# Autodesk Inventor assembly: 組合檔
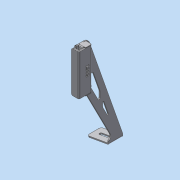
[picture p0: Inventor's stored thumbnail of the model, 180x180]
Saved by Autodesk Inventor 2020 (Build 240168000, 168)
## iProperties
Created: 2015-11-28
Part Number: 組合檔
Document SubType Name: Assembly
Designer: 設計製圖
Author: 設計製圖
## Documents named in this file (13)
- D:\資料庫\設計-3D產品\【May club 】\得利卡-車頂燈架\模型、圖面\車頂燈架-組合 - 複製.iam
- D:\資料庫\設計-3D產品\【May club 】\得利卡-車頂燈架\模型、圖面\吊架-長(R).ipt
- D:\資料庫\設計-3D產品\【May club 】\得利卡-車頂燈架\模型、圖面\概-膠條.ipt
- D:\資料庫\設計-3D產品\【May club 】\得利卡-車頂燈架\模型、圖面\概-泡棉墊(1).ipt
- D:\資料庫\設計-3D產品\【May club 】\得利卡-車頂燈架\模型、圖面\概-泡棉墊(3).ipt
- D:\資料庫\設計-3D產品\【 鐵蹄 】\------鐵蹄工廠素材------ -\拉帽-M8.ipt
- D:\資料庫\設計-3D產品\【May club 】\得利卡-車頂燈架\模型、圖面\焊接組件-1.ipt
- D:\資料庫\設計-3D產品\【May club 】\得利卡-車頂燈架\模型、圖面\焊接組件-3.ipt
- D:\資料庫\設計-3D產品\【May club 】\得利卡-車頂燈架\模型、圖面\概-泡棉墊(2).ipt
- D:\資料庫\設計-3D產品\【May club 】\得利卡-車頂燈架\模型、圖面\焊接組件-2.ipt
- D:\資料庫\設計-3D產品\材料庫\【螺絲】\止付螺絲\止付螺絲-M8-20.ipt
- D:\資料庫\設計-3D產品\【May club 】\得利卡-車頂燈架\模型、圖面\車身圖.ipt
- D:\資料庫\設計-3D產品\【May club 】\得利卡-車頂燈架\模型、圖面\吊架組件-ㄇ槽.ipt
## Components (14 placed, 12 different names)
1. 車身圖:1 — 貼合:33
2. 吊架組件-ㄇ槽:1 — 貼合:6, 齊平:2, 齊平:3, 貼合:8, 齊平:4, 貼合:17, 貼合:18, 貼合:24, 貼合:35, 貼合:36, 貼合:37, 貼合:38
3. 吊架-長(R):1 — 貼合:3, 貼合:4, 齊平:1, 貼合:18, 貼合:23, 貼合:25, 貼合:26, 貼合:28, 齊平:9, 齊平:10, 貼合:33
4. 焊接組件-1:1 — 貼合:29, 貼合:30, 齊平:11
5. 焊接組件-3:1 — 貼合:23, 貼合:24, 貼合:25, 貼合:26, 貼合:27, 齊平:7, 齊平:8
6. 焊接組件-2:1 — 貼合:28, 齊平:9, 齊平:10, 貼合:29, 貼合:30, 齊平:11
7. 拉帽-M8:1 — 齊平:6, 貼合:15, 貼合:17, 貼合:31, 貼合:35, 貼合:37
8. 拉帽-M8:2 — 齊平:6, 貼合:15, 貼合:32, 貼合:36, 貼合:38
9. 概-泡棉墊(2):1 — 貼合:27, 齊平:7, 齊平:8
10. 概-膠條:1 — 貼合:3, 貼合:4, 齊平:1
11. 概-泡棉墊(1):1 — 貼合:6, 齊平:2, 齊平:3, 貼合:9
12. 概-泡棉墊(3):1 — 貼合:8, 貼合:9, 齊平:4
13. 止付螺絲-M8-20:1 — 齊平:12, 貼合:31
14. 止付螺絲-M8-20:2 — 齊平:12, 貼合:32
## Relationships (34: Mate 23, Flush 11)
- 貼合:3 [Mate]: 吊架-長(R):1 ↔ 概-膠條:1
- 貼合:4 [Mate]: 吊架-長(R):1 ↔ 概-膠條:1
- 齊平:1 [Flush]: 吊架-長(R):1 ↔ 概-膠條:1
- 貼合:6 [Mate]: 吊架組件-ㄇ槽:1 ↔ 概-泡棉墊(1):1
- 齊平:2 [Flush]: 吊架組件-ㄇ槽:1 ↔ 概-泡棉墊(1):1
- 齊平:3 [Flush]: 吊架組件-ㄇ槽:1 ↔ 概-泡棉墊(1):1
- 貼合:8 [Mate]: 吊架組件-ㄇ槽:1 ↔ 概-泡棉墊(3):1
- 貼合:9 [Mate]: 概-泡棉墊(1):1 ↔ 概-泡棉墊(3):1
- 齊平:4 [Flush]: 吊架組件-ㄇ槽:1 ↔ 概-泡棉墊(3):1
- 齊平:6 [Flush]: 拉帽-M8:1 ↔ 拉帽-M8:2
- 貼合:15 [Mate]: 拉帽-M8:1 ↔ 拉帽-M8:2
- 貼合:17 [Mate]: 吊架組件-ㄇ槽:1 ↔ 拉帽-M8:1
- 貼合:18 [Mate]: 吊架組件-ㄇ槽:1 ↔ 吊架-長(R):1
- 貼合:23 [Mate]: 吊架-長(R):1 ↔ 焊接組件-3:1
- 貼合:24 [Mate]: 吊架組件-ㄇ槽:1 ↔ 焊接組件-3:1
- 貼合:25 [Mate]: 吊架-長(R):1 ↔ 焊接組件-3:1
- 貼合:26 [Mate]: 吊架-長(R):1 ↔ 焊接組件-3:1
- 貼合:27 [Mate]: 焊接組件-3:1 ↔ 概-泡棉墊(2):1
- 齊平:7 [Flush]: 焊接組件-3:1 ↔ 概-泡棉墊(2):1
- 齊平:8 [Flush]: 焊接組件-3:1 ↔ 概-泡棉墊(2):1
- 貼合:28 [Mate]: 吊架-長(R):1 ↔ 焊接組件-2:1
- 齊平:9 [Flush]: 吊架-長(R):1 ↔ 焊接組件-2:1
- 齊平:10 [Flush] (35 mm): 吊架-長(R):1 ↔ 焊接組件-2:1
- 貼合:29 [Mate]: 焊接組件-1:1 ↔ 焊接組件-2:1
- 貼合:30 [Mate]: 焊接組件-1:1 ↔ 焊接組件-2:1
- 齊平:11 [Flush]: 焊接組件-1:1 ↔ 焊接組件-2:1
- 齊平:12 [Flush]: 止付螺絲-M8-20:1 ↔ 止付螺絲-M8-20:2
- 貼合:31 [Mate]: 拉帽-M8:1 ↔ 止付螺絲-M8-20:1
- 貼合:32 [Mate]: 拉帽-M8:2 ↔ 止付螺絲-M8-20:2
- 貼合:33 [Mate]: 車身圖:1 ↔ 吊架-長(R):1
- 貼合:35 [Mate]: 吊架組件-ㄇ槽:1 ↔ 拉帽-M8:1
- 貼合:36 [Mate]: 吊架組件-ㄇ槽:1 ↔ 拉帽-M8:2
- 貼合:37 [Mate]: 吊架組件-ㄇ槽:1 ↔ 拉帽-M8:1
- 貼合:38 [Mate]: 吊架組件-ㄇ槽:1 ↔ 拉帽-M8:2
